# Autodesk Inventor assembly: OnyxBody
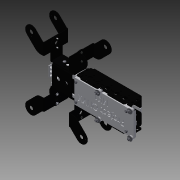
[picture p0: Inventor's stored thumbnail of the model, 180x180]
Saved by Autodesk Inventor 2015 (Build 190159000, 159)
## iProperties
Created: 2015-05-21
Part Number: OnyxBody
Document SubType Name: Assembly
Designer: Quinn
Author: Quinn
## Documents named in this file (15)
- C:\Users\Quinn\Desktop\3DCNC Design\InventorModels\OnyxBody.iam
- C:\Users\Quinn\Desktop\3DCNC Design\InventorModels\Metal\Brackets\asb-12-StandardCChannel.ipt
- C:\Users\Quinn\Desktop\3DCNC Design\InventorModels\Metal\Brackets\asb-06-LTab.ipt
- C:\Users\Quinn\Desktop\3DCNC Design\InventorModels\Metal\Brackets\asb-09-StandardC.ipt
- C:\Users\Quinn\Desktop\3DCNC Design\InventorModels\Metal\Brackets\asb-15-MulitPurpose.ipt
- C:\Users\Quinn\Desktop\3DCNC Design\InventorModels\Plastics\RearCarriageSupport.ipt
- C:\Users\Quinn\Desktop\3DCNC Design\InventorModels\Plastics\RearCarriageCarrierPlate.ipt
- C:\Users\Quinn\Desktop\3DCNC Design\InventorModels\Metal\Brackets\asb-11-angleC.ipt
- C:\Users\Quinn\Desktop\3DCNC Design\InventorModels\Plastics\OnxyBelly.ipt
- C:\Users\Quinn\Desktop\3DCNC Design\InventorModels\Hardware\Screws\2-56 X 0.250 PHS (PHS-02).ipt
- C:\Users\Quinn\Desktop\3DCNC Design\InventorModels\Hardware\Nuts\Nut Hex 2-56 (SN-02).ipt
- C:\Users\Quinn\Desktop\3DCNC Design\InventorModels\Hardware\Screws\M3 X 8 LG PHMS (PHS-00).ipt
- C:\Users\Quinn\Desktop\3DCNC Design\InventorModels\Hardware\Nuts\Nut Hex M3.ipt
- C:\Users\Quinn\Desktop\3DCNC Design\InventorModels\Electronics\ssc-32.ipt
- C:\Users\Quinn\Desktop\3DCNC Design\InventorModels\Hardware\Washers\Washer Flat 3mm.ipt
## Components (53 placed, 14 different names)
1. asb-12-StandardCChannel:1 — Mate:1, Mate:5, Mate:6, Mate:24
2. asb-06-LTab:1 — Mate:1, Mate:2
3. asb-09-StandardC:2 — Mate:2, Mate:3, Mate:4
4. asb-15-MulitPurpose:1 — Mate:4, Mate:7, Mate:8, Insert:15, Insert:17
5. asb-15-MulitPurpose:2 — Mate:3, Insert:14, Insert:16
6. asb-09-StandardC:3 — Mate:5, Mate:11, Mate:12, Insert:2, Insert:3, Insert:4, Insert:5, Insert:6, Insert:7
7. asb-09-StandardC:4 — Mate:6, Mate:9, Mate:10, Mate:23, Insert:1, Insert:8, Insert:9
8. RearCarriageSupport:1 — Mate:7
9. RearCarriageCarrierPlate:1 — Mate:8, Insert:10, Insert:11, Insert:12, Insert:13, Insert:18, Insert:19, Insert:20, Insert:21, Insert:23, Insert:26
10. asb-11-angleC:1 — Mate:11, Mate:17, Mate:18
11. asb-11-angleC:2 — Mate:12, Mate:19, Mate:20
12. asb-11-angleC:3 — Mate:9, Mate:21, Mate:22
13. asb-11-angleC:4 — Mate:10, Mate:15, Mate:16
14. 2-56 X 0.250 PHS (PHS-02):3 — Mate:15
15. 2-56 X 0.250 PHS (PHS-02):4 — Mate:16
16. 2-56 X 0.250 PHS (PHS-02):5 — Mate:17
17. 2-56 X 0.250 PHS (PHS-02):6 — Mate:18
18. 2-56 X 0.250 PHS (PHS-02):7 — Mate:20
19. 2-56 X 0.250 PHS (PHS-02):8 — Mate:22
20. 2-56 X 0.250 PHS (PHS-02):9 — Mate:19
21. 2-56 X 0.250 PHS (PHS-02):10 — Mate:21
22. Nut Hex 2-56 (SN-02):1 — Mate:23
23. Nut Hex 2-56 (SN-02):2 — Insert:1
24. Nut Hex 2-56 (SN-02):3 — Insert:3
25. Nut Hex 2-56 (SN-02):4 — Insert:2
26. Nut Hex 2-56 (SN-02):5 — Insert:4
27. Nut Hex 2-56 (SN-02):6 — Insert:5
28. OnxyBelly:1 — Mate:24
29. M3 X 8 LG PHMS (PHS-00):1 — Insert:6
30. M3 X 8 LG PHMS (PHS-00):2 — Insert:7
31. M3 X 8 LG PHMS (PHS-00):3 — Insert:8
32. M3 X 8 LG PHMS (PHS-00):4 — Insert:9
33. M3 X 8 LG PHMS (PHS-00):5 — Insert:10
34. M3 X 8 LG PHMS (PHS-00):6 — Insert:12
35. M3 X 8 LG PHMS (PHS-00):7 — Insert:11
36. M3 X 8 LG PHMS (PHS-00):8 — Insert:13
37. Nut Hex M3:1 — Insert:17
38. Nut Hex M3:2 — Insert:16
39. Nut Hex M3:3 — Insert:14
40. Nut Hex M3:4 — Insert:15
41. ssc-32:1 — Insert:22, Mate:25, Mate:26, Mate:27, Mate:28
42. Washer Flat 3mm:1 — Insert:19
43. Washer Flat 3mm:2 — Insert:20
44. Washer Flat 3mm:6 — Insert:21
45. Washer Flat 3mm:7 — Insert:18, Insert:22
46. M3 X 8 LG PHMS (PHS-00):9 — Mate:25
47. M3 X 8 LG PHMS (PHS-00):10 — Mate:28, Insert:24
48. M3 X 8 LG PHMS (PHS-00):11 — Mate:26, Insert:25
49. M3 X 8 LG PHMS (PHS-00):12 — Mate:27
50. Nut Hex M3:5 — Insert:25
51. Nut Hex M3:6 — Insert:24
52. Nut Hex M3:7 — Insert:23
53. Nut Hex M3:8 — Insert:26
## Relationships (52: Mate 26, Insert 26)
- Mate:1: asb-12-StandardCChannel:1 ↔ asb-06-LTab:1
- Mate:2: asb-06-LTab:1 ↔ asb-09-StandardC:2
- Mate:3: asb-09-StandardC:2 ↔ asb-15-MulitPurpose:2
- Mate:4: asb-09-StandardC:2 ↔ asb-15-MulitPurpose:1
- Mate:5: asb-12-StandardCChannel:1 ↔ asb-09-StandardC:3
- Mate:6: asb-12-StandardCChannel:1 ↔ asb-09-StandardC:4
- Mate:7: asb-15-MulitPurpose:1 ↔ RearCarriageSupport:1
- Mate:8: asb-15-MulitPurpose:1 ↔ RearCarriageCarrierPlate:1
- Mate:9: asb-09-StandardC:4 ↔ asb-11-angleC:3
- Mate:10: asb-09-StandardC:4 ↔ asb-11-angleC:4
- Mate:11: asb-09-StandardC:3 ↔ asb-11-angleC:1
- Mate:12: asb-09-StandardC:3 ↔ asb-11-angleC:2
- Mate:15: asb-11-angleC:4 ↔ 2-56 X 0.250 PHS (PHS-02):3
- Mate:16: asb-11-angleC:4 ↔ 2-56 X 0.250 PHS (PHS-02):4
- Mate:17: asb-11-angleC:1 ↔ 2-56 X 0.250 PHS (PHS-02):5
- Mate:18: asb-11-angleC:1 ↔ 2-56 X 0.250 PHS (PHS-02):6
- Mate:19: asb-11-angleC:2 ↔ 2-56 X 0.250 PHS (PHS-02):9
- Mate:20: asb-11-angleC:2 ↔ 2-56 X 0.250 PHS (PHS-02):7
- Mate:21: asb-11-angleC:3 ↔ 2-56 X 0.250 PHS (PHS-02):10
- Mate:22: asb-11-angleC:3 ↔ 2-56 X 0.250 PHS (PHS-02):8
- Mate:23: asb-09-StandardC:4 ↔ Nut Hex 2-56 (SN-02):1
- Insert:1: asb-09-StandardC:4 ↔ Nut Hex 2-56 (SN-02):2
- Insert:2: asb-09-StandardC:3 ↔ Nut Hex 2-56 (SN-02):4
- Insert:3: asb-09-StandardC:3 ↔ Nut Hex 2-56 (SN-02):3
- Insert:4: asb-09-StandardC:3 ↔ Nut Hex 2-56 (SN-02):5
- Insert:5: asb-09-StandardC:3 ↔ Nut Hex 2-56 (SN-02):6
- Mate:24: asb-12-StandardCChannel:1 ↔ OnxyBelly:1
- Insert:6: asb-09-StandardC:3 ↔ M3 X 8 LG PHMS (PHS-00):1
- Insert:7: asb-09-StandardC:3 ↔ M3 X 8 LG PHMS (PHS-00):2
- Insert:8: asb-09-StandardC:4 ↔ M3 X 8 LG PHMS (PHS-00):3
- Insert:9: asb-09-StandardC:4 ↔ M3 X 8 LG PHMS (PHS-00):4
- Insert:10: RearCarriageCarrierPlate:1 ↔ M3 X 8 LG PHMS (PHS-00):5
- Insert:11: RearCarriageCarrierPlate:1 ↔ M3 X 8 LG PHMS (PHS-00):7
- Insert:12: RearCarriageCarrierPlate:1 ↔ M3 X 8 LG PHMS (PHS-00):6
- Insert:13: RearCarriageCarrierPlate:1 ↔ M3 X 8 LG PHMS (PHS-00):8
- Insert:14: asb-15-MulitPurpose:2 ↔ Nut Hex M3:3
- Insert:15: asb-15-MulitPurpose:1 ↔ Nut Hex M3:4
- Insert:16: asb-15-MulitPurpose:2 ↔ Nut Hex M3:2
- Insert:17: asb-15-MulitPurpose:1 ↔ Nut Hex M3:1
- Insert:18: RearCarriageCarrierPlate:1 ↔ Washer Flat 3mm:7
- Insert:19: RearCarriageCarrierPlate:1 ↔ Washer Flat 3mm:1
- Insert:20: RearCarriageCarrierPlate:1 ↔ Washer Flat 3mm:2
- Insert:21: RearCarriageCarrierPlate:1 ↔ Washer Flat 3mm:6
- Insert:22: ssc-32:1 ↔ Washer Flat 3mm:7
- Mate:25: ssc-32:1 ↔ M3 X 8 LG PHMS (PHS-00):9
- Mate:26: ssc-32:1 ↔ M3 X 8 LG PHMS (PHS-00):11
- Mate:27: ssc-32:1 ↔ M3 X 8 LG PHMS (PHS-00):12
- Mate:28: ssc-32:1 ↔ M3 X 8 LG PHMS (PHS-00):10
- Insert:23: RearCarriageCarrierPlate:1 ↔ Nut Hex M3:7
- Insert:24: M3 X 8 LG PHMS (PHS-00):10 ↔ Nut Hex M3:6
- Insert:25: M3 X 8 LG PHMS (PHS-00):11 ↔ Nut Hex M3:5
- Insert:26: RearCarriageCarrierPlate:1 ↔ Nut Hex M3:8
